# Autodesk Inventor assembly: Main Assembly
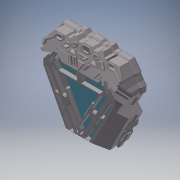
[picture p0: Inventor's stored thumbnail of the model, 180x180]
Saved by Autodesk Inventor 2017 (Build 210142000, 142)
## iProperties
Created: 2019-07-27
Part Number: Main Assembly
Document SubType Name: Assembly
Designer: Mitch
Author: Mitch
## Documents named in this file (9)
- E:\Youtube Channel\Pojects\Iron Man arc reactor\MECH\Main Assembly.iam
- E:\Youtube Channel\Pojects\Iron Man arc reactor\MECH\BackPlate.ipt
- E:\Youtube Channel\Pojects\Iron Man arc reactor\MECH\ElectronicsTray.ipt
- E:\Youtube Channel\Pojects\Iron Man arc reactor\MECH\LightScreen.ipt
- E:\Youtube Channel\Pojects\Iron Man arc reactor\MECH\FrontPlate.ipt
- E:\Youtube Channel\Pojects\Iron Man arc reactor\MECH\LED_Board.ipt
- E:\Youtube Channel\Pojects\Iron Man arc reactor\MECH\LIPO.ipt
- E:\Youtube Channel\Pojects\Iron Man arc reactor\MECH\microB.ipt
- E:\Youtube Channel\Pojects\Iron Man arc reactor\MECH\femaleThruHoleUSB.ipt
## Components (8 placed, 8 different names)
1. BackPlate:1 — Mate:1, Mate:2, Mate:3, Flush:1
2. ElectronicsTray:1 — Mate:1, Mate:2, Mate:3, Mate:4, Mate:10, Mate:11, Mate:12, Mate:13, Mate:14, Flush:3, Mate:15, Mate:16, Mate:18, Mate:19
3. LightScreen:1 — Mate:7, Mate:8, Mate:9
4. FrontPlate:1 — Mate:7, Mate:8, Mate:9, Mate:10, Mate:11
5. LED_Board:1 — Mate:4, Flush:1, Mate:6
6. LIPO:1 — Mate:12, Mate:13
7. microB:1 — Mate:14, Flush:3, Mate:15
8. femaleThruHoleUSB:1 — Mate:16, Mate:18, Mate:19
## Relationships (20: Mate 17, Flush 3)
- Mate:1: BackPlate:1 ↔ ElectronicsTray:1
- Mate:2 (0.9525 mm): BackPlate:1 ↔ ElectronicsTray:1
- Mate:3 (0.8001 mm): BackPlate:1 ↔ ElectronicsTray:1
- Mate:4: ElectronicsTray:1 ↔ LED_Board:1
- Flush:1 (31.1658 mm): BackPlate:1 ↔ LED_Board:1
- Flush:2 (-70.358 mm)
- Mate:6 (32.385 mm): LED_Board:1
- Mate:7: LightScreen:1 ↔ FrontPlate:1
- Mate:8 (0.3175 mm): LightScreen:1 ↔ FrontPlate:1
- Mate:9 (0.3556 mm): LightScreen:1 ↔ FrontPlate:1
- Mate:10: ElectronicsTray:1 ↔ FrontPlate:1
- Mate:11 (-5.969 mm): ElectronicsTray:1 ↔ FrontPlate:1
- Mate:12: ElectronicsTray:1 ↔ LIPO:1
- Mate:13: ElectronicsTray:1 ↔ LIPO:1
- Mate:14: ElectronicsTray:1 ↔ microB:1
- Flush:3: ElectronicsTray:1 ↔ microB:1
- Mate:15: ElectronicsTray:1 ↔ microB:1
- Mate:16 (-13.8938 mm): ElectronicsTray:1 ↔ femaleThruHoleUSB:1
- Mate:18: ElectronicsTray:1 ↔ femaleThruHoleUSB:1
- Mate:19: ElectronicsTray:1 ↔ femaleThruHoleUSB:1
